# Autodesk Inventor assembly: Tiger
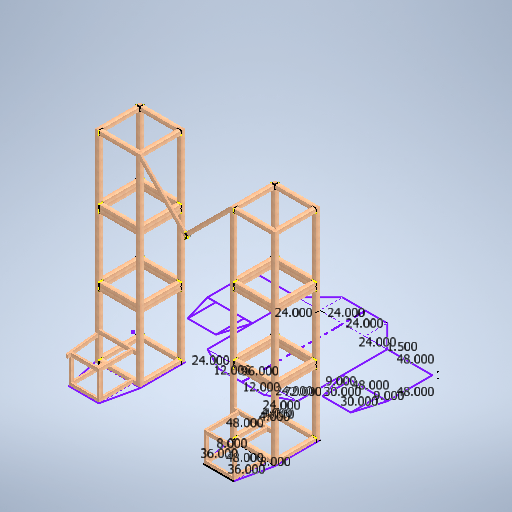
[picture p0: Inventor's stored thumbnail of the model, 512x512]
Saved by Autodesk Inventor 2025 (Build 290162000, 162)
## iProperties
Created: 2024-06-05
Part Number: Tiger
Document SubType Name: Assembly
Designer: Cupri
Mass: 180546 g
Surface Area: 136258 cm^2
Volume: 328266 cm^3
Density: 0.55 g/cm^3
Author: Cupri
## Documents named in this file (15)
- C:\Users\Cupri\OneDrive\Documents\TigerBurn\USCTigerBurn24\v1\Tiger.iam
- C:\Users\Cupri\OneDrive\Documents\TigerBurn\USCTigerBurn24\Standard Timber\4x4x72.ipt
- C:\Users\Cupri\OneDrive\Documents\TigerBurn\USCTigerBurn24\Standard Timber\4x4x40.ipt
- C:\Users\Cupri\OneDrive\Documents\TigerBurn\USCTigerBurn24\Standard Timber\2x4x36.ipt
- C:\Users\Cupri\OneDrive\Documents\TigerBurn\USCTigerBurn24\Standard Timber\2x4x40.ipt
- C:\Users\Cupri\OneDrive\Documents\TigerBurn\USCTigerBurn24\Standard Timber\2x4x24.ipt
- C:\Users\Cupri\OneDrive\Documents\TigerBurn\USCTigerBurn24\Standard Timber\2x4x28.ipt
- C:\Users\Cupri\OneDrive\Documents\TigerBurn\USCTigerBurn24\Standard Timber\2x4x72 (45 90).ipt
- C:\Users\Cupri\OneDrive\Documents\TigerBurn\USCTigerBurn24\Standard Timber\2x4x68 (45 90).ipt
- C:\Users\Cupri\OneDrive\Documents\TigerBurn\USCTigerBurn24\v1\Tiger\AIP\FEA\epzzwi8io.fins
- C:\Users\Cupri\OneDrive\Documents\TigerBurn\USCTigerBurn24\v1\Tiger\AIP\FEA\epzzwi8io.fsat
- C:\Users\Cupri\OneDrive\Documents\TigerBurn\USCTigerBurn24\v1\Tiger\AIP\FEA\epzzwi8io.ftes
- C:\Users\Cupri\OneDrive\Documents\TigerBurn\USCTigerBurn24\v1\Tiger\AIP\FEA\epzzwi8io.fwiz
- C:\Users\Cupri\OneDrive\Documents\TigerBurn\USCTigerBurn24\v1\Tiger\AIP\FEA\epzzwi8jk.fmsh
- C:\Users\Cupri\OneDrive\Documents\TigerBurn\USCTigerBurn24\v1\Tiger\AIP\FEA\epzzwi8jl.fres
## Components (92 placed, 8 different names)
1. 2x4x72 (45 90):1 — Mate:37, Flush:40, Rigid:104
2. 2x4x68 (45 90):1 — Mate:38, Flush:41, Rigid:105
3. 4x4x72:1 — Rigid:1, Rigid:3, Rigid:10, Rigid:11, Flush:39
4. 4x4x72:2 — Rigid:2, Rigid:4, Rigid:8
5. 4x4x40:1 — Rigid:1, Rigid:2
6. 4x4x40:2 — Rigid:3, Rigid:5, Flush:38, Mate:36
7. 4x4x40:3 — Rigid:6, Mate:5, Mate:6, Flush:4, Flush:5, Flush:19, Flush:20
8. 4x4x40:4 — Rigid:4, Rigid:7
9. 4x4x40:5 — Rigid:8
10. 4x4x40:6 — Rigid:9, Rigid:23
11. 4x4x40:7 — Rigid:11
12. 4x4x40:8 — Rigid:10
13. 4x4x72:3 — Rigid:5, Rigid:6, Rigid:9, Mate:4, Flush:3
14. 4x4x72:4 — Rigid:7, Mate:7, Flush:21, Flush:22
15. 4x4x72:5
16. 4x4x72:6
17. 4x4x40:9
18. 4x4x40:10
19. 4x4x40:11 — Rigid:23
20. 4x4x40:12
21. 4x4x40:13
22. 4x4x40:14
23. 4x4x40:15 — Flush:16
24. 4x4x40:16 — Flush:15
25. 4x4x72:7 — Mate:25
26. 4x4x72:8
27. 2x4x40:1 — Mate:4, Flush:3, Mate:5, Mate:8, Flush:6, Mate:9, Flush:7, Flush:17, Flush:18
28. 2x4x36:1 — Mate:6, Flush:4, Rigid:24, Flush:19, Flush:23
29. 2x4x36:2 — Mate:8, Flush:6, Flush:17, Mate:26
30. 2x4x36:3 — Mate:9, Flush:7, Mate:10, Rigid:26, Flush:18, Flush:21
31. 2x4x36:4 — Mate:7, Flush:5, Mate:10, Rigid:25, Rigid:27, Flush:20, Flush:22
32. 2x4x24:1 — Rigid:24
33. 2x4x24:2 — Rigid:25
34. 2x4x28:1 — Rigid:26, Mate:26
35. 2x4x28:2 — Rigid:27, Flush:23
36. 4x4x72:17
37. 4x4x72:18
38. 4x4x40:33 — Flush:16
39. 4x4x40:34 — Flush:15
40. 4x4x40:35
41. 4x4x40:36
42. 4x4x40:37
43. 4x4x40:38
44. 4x4x40:39
45. 4x4x40:40
46. 4x4x72:19 — Mate:25, Mate:38, Flush:41, Rigid:105
47. 4x4x72:20
48. 4x4x72:21
49. 4x4x72:22 — Flush:39
50. 4x4x40:41
51. 4x4x40:42
52. 4x4x40:43
53. 4x4x40:44 — Flush:38, Mate:36
54. 4x4x40:45
55. 4x4x40:46
56. 4x4x40:47
57. 4x4x40:48
58. 4x4x72:23
59. 4x4x72:24
60. 4x4x72:25
61. 4x4x72:26
62. 4x4x40:49
63. 4x4x40:50
64. 4x4x40:51
65. 4x4x40:52
66. 4x4x40:53
67. 4x4x40:54
68. 4x4x40:55
69. 4x4x40:56
70. 4x4x72:27
71. 4x4x72:28
72. 2x4x40:2
73. 2x4x36:5
74. 2x4x36:6
75. 2x4x36:7
76. 2x4x36:8
77. 2x4x24:3
78. 2x4x24:4
79. 2x4x28:3
80. 2x4x28:4
81. 4x4x72:29
82. 4x4x72:30
83. 4x4x40:57
84. 4x4x40:58
85. 4x4x40:59
86. 4x4x40:60
87. 4x4x40:61
88. 4x4x40:62
89. 4x4x40:63
90. 4x4x40:64
91. 4x4x72:31
92. 4x4x72:32 — Mate:37, Flush:40, Rigid:104
## Relationships (131: WeldJoint 78, Flush 32, Mate 21)
- Rigid:1 [WeldJoint]: 4x4x72:1 ↔ 4x4x40:1
- Rigid:2 [WeldJoint]: 4x4x72:2 ↔ 4x4x40:1
- Rigid:3 [WeldJoint]: 4x4x72:1 ↔ 4x4x40:2
- Rigid:4 [WeldJoint]: 4x4x72:2 ↔ 4x4x40:4
- Rigid:5 [WeldJoint]: 4x4x40:2 ↔ 4x4x72:3
- Rigid:6 [WeldJoint]: 4x4x40:3 ↔ 4x4x72:3
- Rigid:7 [WeldJoint]: 4x4x40:4 ↔ 4x4x72:4
- Rigid:8 [WeldJoint]: 4x4x72:2 ↔ 4x4x40:5
- Rigid:9 [WeldJoint]: 4x4x40:6 ↔ 4x4x72:3
- Rigid:10 [WeldJoint]: 4x4x72:1 ↔ 4x4x40:8
- Rigid:11 [WeldJoint]: 4x4x72:1 ↔ 4x4x40:7
- [WeldJoint]: 4x4x72:5 ↔ 4x4x40:9
- [WeldJoint]: 4x4x72:6 ↔ 4x4x40:9
- [WeldJoint]: 4x4x72:5 ↔ 4x4x40:10
- [WeldJoint]: 4x4x72:6 ↔ 4x4x40:12
- [WeldJoint]: 4x4x40:10 ↔ 4x4x72:7
- [WeldJoint]: 4x4x40:11 ↔ 4x4x72:7
- [WeldJoint]: 4x4x40:12 ↔ 4x4x72:8
- [WeldJoint]: 4x4x72:6 ↔ 4x4x40:13
- [WeldJoint]: 4x4x40:14 ↔ 4x4x72:7
- [WeldJoint]: 4x4x72:5 ↔ 4x4x40:16
- [WeldJoint]: 4x4x72:5 ↔ 4x4x40:15
- Rigid:23 [WeldJoint]: 4x4x40:6 ↔ 4x4x40:11
- Mate:4: 4x4x72:3 ↔ 2x4x40:1
- Flush:3: 4x4x72:3 ↔ 2x4x40:1
- Mate:5 (609.6 mm): 4x4x40:3 ↔ 2x4x40:1
- Mate:6 (101.6 mm): 4x4x40:3 ↔ 2x4x36:1
- Flush:4: 4x4x40:3 ↔ 2x4x36:1
- Mate:7 (101.6 mm): 4x4x72:4 ↔ 2x4x36:4
- Flush:5: 4x4x40:3 ↔ 2x4x36:4
- Mate:8 (101.6 mm): 2x4x40:1 ↔ 2x4x36:2
- Flush:6: 2x4x40:1 ↔ 2x4x36:2
- Mate:9: 2x4x40:1 ↔ 2x4x36:3
- Flush:7: 2x4x40:1 ↔ 2x4x36:3
- Mate:10: 2x4x36:3 ↔ 2x4x36:4
- Rigid:24 [WeldJoint]: 2x4x36:1 ↔ 2x4x24:1
- Rigid:25 [WeldJoint]: 2x4x36:4 ↔ 2x4x24:2
- Rigid:26 [WeldJoint]: 2x4x36:3 ↔ 2x4x28:1
- Rigid:27 [WeldJoint]: 2x4x36:4 ↔ 2x4x28:2
- [WeldJoint]: 4x4x72:17 ↔ 4x4x40:33
- [WeldJoint]: 4x4x72:18 ↔ 4x4x40:33
- [WeldJoint]: 4x4x72:17 ↔ 4x4x40:34
- [WeldJoint]: 4x4x72:18 ↔ 4x4x40:36
- [WeldJoint]: 4x4x40:34 ↔ 4x4x72:19
- [WeldJoint]: 4x4x40:35 ↔ 4x4x72:19
- [WeldJoint]: 4x4x40:36 ↔ 4x4x72:20
- [WeldJoint]: 4x4x72:18 ↔ 4x4x40:37
- [WeldJoint]: 4x4x40:38 ↔ 4x4x72:19
- [WeldJoint]: 4x4x72:17 ↔ 4x4x40:40
- [WeldJoint]: 4x4x72:17 ↔ 4x4x40:39
- Mate:25: 4x4x72:7 ↔ 4x4x72:19
- Flush:15: 4x4x40:16 ↔ 4x4x40:34
- Flush:16: 4x4x40:15 ↔ 4x4x40:33
- Flush:17: 2x4x40:1 ↔ 2x4x36:2
- Flush:18: 2x4x40:1 ↔ 2x4x36:3
- Flush:19: 4x4x40:3 ↔ 2x4x36:1
- Flush:20: 4x4x40:3 ↔ 2x4x36:4
- Flush:21 (203.2 mm): 4x4x72:4 ↔ 2x4x36:3
- Flush:22 (203.2 mm): 4x4x72:4 ↔ 2x4x36:4
- Flush:23: 2x4x36:1 ↔ 2x4x28:2
- Mate:26: 2x4x36:2 ↔ 2x4x28:1
- [WeldJoint]: 4x4x72:21 ↔ 4x4x40:41
- [WeldJoint]: 4x4x72:22 ↔ 4x4x40:41
- [WeldJoint]: 4x4x72:21 ↔ 4x4x40:42
- [WeldJoint]: 4x4x72:22 ↔ 4x4x40:44
- [WeldJoint]: 4x4x40:42 ↔ 4x4x72:23
- [WeldJoint]: 4x4x40:43 ↔ 4x4x72:23
- [WeldJoint]: 4x4x40:44 ↔ 4x4x72:24
- [WeldJoint]: 4x4x72:22 ↔ 4x4x40:45
- [WeldJoint]: 4x4x40:46 ↔ 4x4x72:23
- [WeldJoint]: 4x4x72:21 ↔ 4x4x40:48
- [WeldJoint]: 4x4x72:21 ↔ 4x4x40:47
- [WeldJoint]: 4x4x72:25 ↔ 4x4x40:49
- [WeldJoint]: 4x4x72:26 ↔ 4x4x40:49
- [WeldJoint]: 4x4x72:25 ↔ 4x4x40:50
- [WeldJoint]: 4x4x72:26 ↔ 4x4x40:52
- [WeldJoint]: 4x4x40:50 ↔ 4x4x72:27
- [WeldJoint]: 4x4x40:51 ↔ 4x4x72:27
- [WeldJoint]: 4x4x40:52 ↔ 4x4x72:28
- [WeldJoint]: 4x4x72:26 ↔ 4x4x40:53
- [WeldJoint]: 4x4x40:54 ↔ 4x4x72:27
- [WeldJoint]: 4x4x72:25 ↔ 4x4x40:56
- [WeldJoint]: 4x4x72:25 ↔ 4x4x40:55
- [WeldJoint]: 4x4x40:46 ↔ 4x4x40:51
- [Mate]: 4x4x72:23 ↔ 2x4x40:2
- [Flush]: 4x4x72:23 ↔ 2x4x40:2
- [Mate] (609.6 mm): 4x4x40:43 ↔ 2x4x40:2
- [Mate] (101.6 mm): 4x4x40:43 ↔ 2x4x36:5
- [Flush]: 4x4x40:43 ↔ 2x4x36:5
- [Mate] (101.6 mm): 4x4x72:24 ↔ 2x4x36:8
- [Flush]: 4x4x40:43 ↔ 2x4x36:8
- [Mate] (101.6 mm): 2x4x40:2 ↔ 2x4x36:6
- [Flush]: 2x4x40:2 ↔ 2x4x36:6
- [Mate]: 2x4x40:2 ↔ 2x4x36:7
- [Flush]: 2x4x40:2 ↔ 2x4x36:7
- [Mate]: 2x4x36:7 ↔ 2x4x36:8
- [WeldJoint]: 2x4x36:5 ↔ 2x4x24:3
- [WeldJoint]: 2x4x36:8 ↔ 2x4x24:4
- [WeldJoint]: 2x4x36:7 ↔ 2x4x28:3
- [WeldJoint]: 2x4x36:8 ↔ 2x4x28:4
- [WeldJoint]: 4x4x72:29 ↔ 4x4x40:57
- [WeldJoint]: 4x4x72:30 ↔ 4x4x40:57
- [WeldJoint]: 4x4x72:29 ↔ 4x4x40:58
- [WeldJoint]: 4x4x72:30 ↔ 4x4x40:60
- [WeldJoint]: 4x4x40:58 ↔ 4x4x72:31
- [WeldJoint]: 4x4x40:59 ↔ 4x4x72:31
- [WeldJoint]: 4x4x40:60 ↔ 4x4x72:32
- [WeldJoint]: 4x4x72:30 ↔ 4x4x40:61
- [WeldJoint]: 4x4x40:62 ↔ 4x4x72:31
- [WeldJoint]: 4x4x72:29 ↔ 4x4x40:64
- [WeldJoint]: 4x4x72:29 ↔ 4x4x40:63
- [Mate]: 4x4x72:27 ↔ 4x4x72:31
- [Flush]: 4x4x40:56 ↔ 4x4x40:58
- [Flush]: 4x4x40:55 ↔ 4x4x40:57
- [Flush]: 2x4x40:2 ↔ 2x4x36:6
- [Flush]: 2x4x40:2 ↔ 2x4x36:7
- [Flush]: 4x4x40:43 ↔ 2x4x36:5
- [Flush]: 4x4x40:43 ↔ 2x4x36:8
- [Flush] (203.2 mm): 4x4x72:24 ↔ 2x4x36:7
- [Flush] (203.2 mm): 4x4x72:24 ↔ 2x4x36:8
- [Flush]: 2x4x36:5 ↔ 2x4x28:4
- [Mate]: 2x4x36:6 ↔ 2x4x28:3
- Flush:38: 4x4x40:2 ↔ 4x4x40:44
- Flush:39: 4x4x72:1 ↔ 4x4x72:22
- Mate:36 (2438.4 mm): 4x4x40:2 ↔ 4x4x40:44
- Mate:37: 2x4x72 (45 90):1 ↔ 4x4x72:32
- Flush:40: 2x4x72 (45 90):1 ↔ 4x4x72:32
- Rigid:104 [WeldJoint]: 2x4x72 (45 90):1 ↔ 4x4x72:32
- Mate:38: 2x4x68 (45 90):1 ↔ 4x4x72:19
- Flush:41: 2x4x68 (45 90):1 ↔ 4x4x72:19
- Rigid:105 [WeldJoint]: 2x4x68 (45 90):1 ↔ 4x4x72:19
## Named parameters: d40_d29 = 0 mm, d41_d30 = 0 mm, d42_d31 = 0 mm, d43_d32 = 0 mm, d44_d33 = 0 mm, d45_d34 = 0 mm, d46_d35 = 0 mm, d47_d36 = 0 mm, d48_d37 = 0 mm, d49_d38 = 0 mm, d50_d39 = 0 mm, sa_0 = 22241.1, d129_d40_d29 = 0 mm, d130_d41_d30 = 0 mm, d131_d42_d31 = 0 mm, d132_d43_d32 = 0 mm, d133_d44_d33 = 0 mm, d134_d45_d34 = 0 mm, d135_d46_d35 = 0 mm, d136_d47_d36 = 0 mm, d137_d48_d37 = 0 mm, d138_d49_d38 = 0 mm, d139_d50_d39 = 0 mm, d151_d141 = 0 mm, d152_d142 = 0 mm, d153_d143 = 0 mm, d154_d144 = 0 mm, d155_d145 = 0 mm, d156_d146 = 0 mm, d157_d147 = 203.2 mm, d158_d148 = 203.2 mm, d159_d149 = 0 mm, d160_d150 = 0 mm, d161_d129_d40_d29 = 0 mm, d162_d130_d41_d30 = 0 mm, d163_d131_d42_d31 = 0 mm, d164_d132_d43_d32 = 0 mm, d165_d133_d44_d33 = 0 mm, d166_d134_d45_d34 = 0 mm, d167_d135_d46_d35 = 0 mm, d168_d136_d47_d36 = 0 mm, d169_d137_d48_d37 = 0 mm, d170_d138_d49_d38 = 0 mm, d171_d139_d50_d39 = 0 mm, d172_d140 = 0 mm, d173_d61 = 0 mm, d174_d62 = 0 mm, d175_d63 = 609.6 mm, d176_d68 = 101.6 mm, d177_d69 = 0 mm, d178_d70 = 101.6 mm, d179_d71 = 0 mm, d180_d72 = 101.6 mm, d181_d73 = 0 mm, d182_d74 = 0 mm, d183_d75 = 0 mm, d184_d76 = 0 mm, d185_d77 = 0 mm, d186_d78 = 0 mm, d187_d79 = 0 mm, d188_d80 = 0 mm, d189_d51 = 0 mm, d190_d31 = 0 mm, d191_d32 = 0 mm, d192_d33 = 0 mm, d193_d34 = 0 mm, d194_d35 = 0 mm, d195_d36 = 0 mm, d196_d37 = 0 mm, d197_d38 = 0 mm, d198_d39 = 0 mm, d199_d40_d29 = 0 mm, d200_d41_d30 = 0 mm, d201_d42_d31 = 0 mm, d202_d43_d32 = 0 mm, d203_d44_d33 = 0 mm, d204_d45_d34 = 0 mm, d205_d46_d35 = 0 mm, d206_d47_d36 = 0 mm, d207_d48_d37 = 0 mm, d208_d49_d38 = 0 mm, d209_d50_d39 = 0 mm, d210_d29 = 0 mm, d211_d30 = 0 mm
note: some values were not read from the file. Shown as the stored number, unit unknown: "sa_0".
